# Autodesk Inventor assembly: ChipHolder
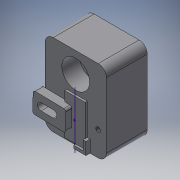
[picture p0: Inventor's stored thumbnail of the model, 180x180]
Saved by Autodesk Inventor 2019 (Build 230136000, 136)
## iProperties
Created: 2019-08-13
Part Number: ChipHolder
Document SubType Name: Assembly
Designer: aorfi
Author: aorfi
## Documents named in this file (4)
- C:\Users\aorfi\Documents\IQC\CustomParts\ChipHolder.iam
- C:\Users\aorfi\Documents\IQC\CustomParts\ChipHolder.ipt
- C:\Users\aorfi\Documents\IQC\CustomParts\RubayetChip.ipt
- C:\Users\aorfi\Documents\IQC\CustomParts\ChipClip.ipt
## Components (3 placed, 3 different names)
1. ChipHolder:1 — Mate:1, Mate:2, Flush:1, Mate:3, Mate:6, Mate:7, Mate:9
2. RubayetChip:1 — Mate:3, Mate:6, Mate:7
3. ChipClip:1 — Mate:9
## Relationships (7: Mate 6, Flush 1)
- Mate:1: ChipHolder:1
- Mate:2: ChipHolder:1
- Flush:1: ChipHolder:1
- Mate:3: ChipHolder:1 ↔ RubayetChip:1
- Mate:6: ChipHolder:1 ↔ RubayetChip:1
- Mate:7: ChipHolder:1 ↔ RubayetChip:1
- Mate:9: ChipHolder:1 ↔ ChipClip:1
